# Autodesk Inventor assembly: CombinedScreenHolder
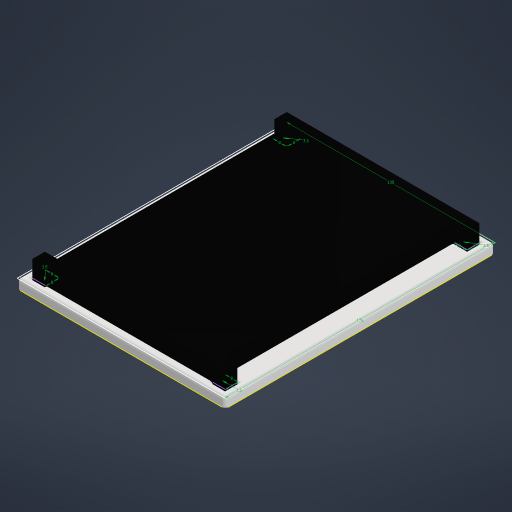
[picture p0: Inventor's stored thumbnail of the model, 512x512]
Saved by Autodesk Inventor 2023 (Build 270158000, 158)
## iProperties
Created: 2023-02-22
Part Number: CombinedScreenHolder
Document SubType Name: Assembly
Designer: uzair
Author: uzair
## Documents named in this file (3)
- C:\Users\uzair\Programming\Capstone-MJ02\documentation\3D Models\CombinedScreenHolder.iam
- C:\Users\uzair\Programming\Capstone-MJ02\documentation\3D Models\7InchScreen.ipt
- C:\Users\uzair\Programming\Capstone-MJ02\documentation\3D Models\ScreenHolderBasse.ipt
## Components (2 placed, 2 different names)
1. 7InchScreen:1 — Mate:1, Mate:2, Mate:3
2. ScreenHolderBasse:1 — Mate:1, Mate:2, Mate:3
## Relationships (3: Mate 3)
- Mate:1: 7InchScreen:1 ↔ ScreenHolderBasse:1
- Mate:2: 7InchScreen:1 ↔ ScreenHolderBasse:1
- Mate:3: 7InchScreen:1 ↔ ScreenHolderBasse:1
